# Autodesk Inventor assembly: 4_right_leg_true_final
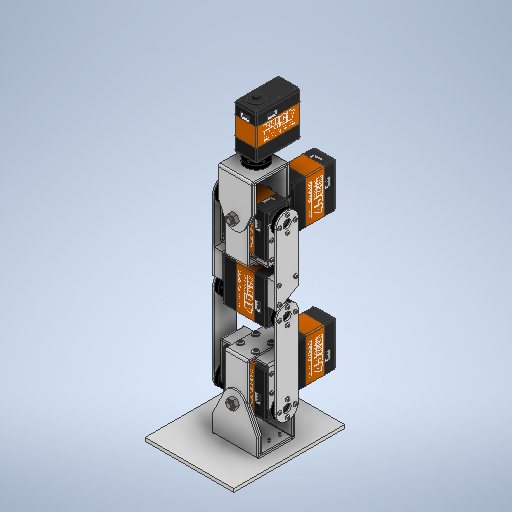
[picture p0: Inventor's stored thumbnail of the model, 512x512]
Saved by Autodesk Inventor 2026.1 (Build 301233000, 233)
## iProperties
Created: 2025-08-13
Part Number: 4_right_leg_true_final
Document SubType Name: Assembly
Designer: User
Author: User
## Documents named in this file (28)
- C:\Users\User\Documents\The Maverick's Files\College 3-3\로보인 프로젝트\RHp_Humanoid_ver1\Assembly\4_right_leg_true_final.iam
- C:\Users\User\Documents\The Maverick's Files\College 3-3\로보인 프로젝트\RHp_Humanoid_ver1\Part\HTD-45H, Horn\HTD-45H\HTD-45H.iam
- C:\Users\User\Documents\The Maverick's Files\College 3-3\로보인 프로젝트\RHp_Humanoid_ver1\Part\HTD-45H, Horn\Horn\Top Horn.ipt
- C:\Users\User\Documents\The Maverick's Files\College 3-3\로보인 프로젝트\RHp_Humanoid_ver1\Part\HTD-45H, Horn\Horn\Bottom Horn.ipt
- C:\Users\User\Documents\The Maverick's Files\College 3-3\로보인 프로젝트\RHp_Humanoid_ver1\Part\Frame\Leg\Right Leg\axis_7_supplement_frame.ipt
- C:\Users\User\Documents\The Maverick's Files\College 3-3\로보인 프로젝트\RHp_Humanoid_ver1\Part\Frame\Leg\Right Leg\axis_7_top_frame.ipt
- C:\Users\User\Documents\The Maverick's Files\College 3-3\로보인 프로젝트\RHp_Humanoid_ver1\Part\Frame\Leg\Right Leg\axis_8_bottom_frame.ipt
- C:\Users\User\Documents\The Maverick's Files\College 3-3\로보인 프로젝트\RHp_Humanoid_ver1\Part\Frame\Leg\Right Leg\axis_8_10_connector_frame_non_powered.ipt
- C:\Users\User\Documents\The Maverick's Files\College 3-3\로보인 프로젝트\RHp_Humanoid_ver1\Part\Frame\Leg\Right Leg\axis_8_10_connector_frame_powered.ipt
- C:\Users\User\Documents\The Maverick's Files\College 3-3\로보인 프로젝트\RHp_Humanoid_ver1\Part\Frame\Leg\Right Leg\axis_9_bottom_frame.ipt
- C:\Users\User\Documents\The Maverick's Files\College 3-3\로보인 프로젝트\RHp_Humanoid_ver1\Part\Frame\Leg\3D_printed_part_non_powered.ipt
- C:\Users\User\Documents\The Maverick's Files\College 3-3\로보인 프로젝트\RHp_Humanoid_ver1\Part\Frame\Leg\3D_printed_part_powered.ipt
- C:\Users\User\Documents\The Maverick's Files\College 3-3\로보인 프로젝트\RHp_Humanoid_ver1\Part\Frame\Leg\Right Leg\axis_10_11_connector_frame_non_powered.ipt
- C:\Users\User\Documents\The Maverick's Files\College 3-3\로보인 프로젝트\RHp_Humanoid_ver1\Part\Frame\Leg\Right Leg\axis_10_11_connector_frame_powered.ipt
- C:\Users\User\Documents\The Maverick's Files\College 3-3\로보인 프로젝트\RHp_Humanoid_ver1\Part\Frame\Leg\Right Leg\axis_11_top_frame.ipt
- C:\Users\User\Documents\The Maverick's Files\College 3-3\로보인 프로젝트\RHp_Humanoid_ver1\Part\Frame\Leg\Right Leg\axis_12_top_frame.ipt
- C:\Users\User\Documents\The Maverick's Files\College 3-3\로보인 프로젝트\RHp_Humanoid_ver1\Part\Frame\Leg\Right Leg\axis_12_bottom_frame(top).ipt
- C:\Users\User\Documents\The Maverick's Files\College 3-3\로보인 프로젝트\RHp_Humanoid_ver1\Part\Frame\Leg\Right Leg\axis_12_supplement_frame.ipt
- C:\Users\User\Documents\The Maverick's Files\College 3-3\로보인 프로젝트\RHp_Humanoid_ver1\Part\Frame\Leg\Right Leg\axis_12_bottom_frame(bottom).ipt
- C:\Users\User\Documents\The Maverick's Files\College 3-3\로보인 프로젝트\RHp_Humanoid_ver1\Part\Bolt, Bearing, Nut, Washer\볼트, 너트\볼트, 너트\M2x8접시.ipt
- C:\Users\User\Documents\The Maverick's Files\College 3-3\로보인 프로젝트\RHp_Humanoid_ver1\Part\Bolt, Bearing, Nut, Washer\볼트, 너트\볼트, 너트\M5x10 Bolt.ipt
- C:\Users\User\Documents\The Maverick's Files\College 3-3\로보인 프로젝트\RHp_Humanoid_ver1\Part\Bolt, Bearing, Nut, Washer\볼트, 너트\볼트, 너트\M5 Nylon Nut.ipt
- C:\Users\User\Documents\The Maverick's Files\College 3-3\로보인 프로젝트\RHp_Humanoid_ver1\Part\Bolt, Bearing, Nut, Washer\볼트, 너트\볼트, 너트\M3x6 Bolt.ipt
- C:\Users\User\Documents\The Maverick's Files\College 3-3\로보인 프로젝트\RHp_Humanoid_ver1\Part\Bolt, Bearing, Nut, Washer\볼트, 너트\볼트, 너트\M3 Nut.ipt
- C:\Users\User\Documents\The Maverick's Files\College 3-3\로보인 프로젝트\RHp_Humanoid_ver1\Part\Bolt, Bearing, Nut, Washer\볼트, 너트\볼트, 너트\M2x45 Bolt.ipt
- C:\Users\User\Documents\The Maverick's Files\College 3-3\로보인 프로젝트\RHp_Humanoid_ver1\Part\Bolt, Bearing, Nut, Washer\볼트, 너트\볼트, 너트\M2x12 Bolt.ipt
- C:\Users\User\Documents\The Maverick's Files\College 3-3\로보인 프로젝트\RHp_Humanoid_ver1\Part\Bolt, Bearing, Nut, Washer\볼트, 너트\볼트, 너트\M2x6 Bolt.ipt
- C:\Users\User\Documents\The Maverick's Files\College 3-3\로보인 프로젝트\RHp_Humanoid_ver1\Part\Bolt, Bearing, Nut, Washer\볼트, 너트\볼트, 너트\M2x4 Bolt.ipt
## Components (128 placed, 27 different names)
1. HTD-45H:1 [sub-assembly] — Rotational:1
2. Top Horn:1 — Rotational:1, Rigid:1
3. axis_7_top_frame:1 — Rigid:1, Rigid:2, Rigid:4, Rigid:31
4. axis_7_supplement_frame:1 — Rigid:2, Rigid:29, Rigid:89, Rigid:90, Rigid:91, Rigid:92, Rigid:93, Rigid:94, Rigid:95, Rigid:96
5. HTD-45H:2 [sub-assembly] — Rotational:2, Rigid:3
6. Top Horn:2 — Rigid:7
7. Bottom Horn:2 — Rotational:2, Rigid:8
8. axis_8_bottom_frame:1 — Rigid:3, Rigid:6, Rigid:37, Rigid:38, Rigid:39, Rigid:40, Rigid:71, Rigid:72, Rigid:73, Rigid:74, Rigid:75, Rigid:76, Rigid:77, Rigid:78, Rigid:79
9. axis_8_10_connector_frame_powered:1 — Rigid:7, Rigid:9, Rigid:49, Rigid:50, Rigid:51, Rigid:52, Rigid:53, Rigid:105, Rigid:106, Rigid:107, Rigid:108
10. axis_8_10_connector_frame_non_powered:1 — Rigid:8, Rigid:10, Rigid:54, Rigid:55, Rigid:56, Rigid:113, Rigid:114, Rigid:115, Rigid:116
11. HTD-45H:3 [sub-assembly] — Rotational:5, Rigid:5
12. Top Horn:3 — Rotational:5, Rigid:4
13. axis_9_bottom_frame:1 — Rigid:5, Rigid:6, Rigid:45, Rigid:46, Rigid:47, Rigid:48, Rigid:80, Rigid:81, Rigid:82, Rigid:83, Rigid:84
14. HTD-45H:4 [sub-assembly] — Rotational:6, Rotational:7, Rigid:11, Rigid:12
15. Top Horn:4 — Rotational:7, Rigid:13
16. Bottom Horn:4 — Rotational:6, Rigid:14
17. 3D_printed_part_powered:1 — Rigid:9, Rigid:11
18. 3D_printed_part_non_powered:1 — Rigid:10, Rigid:12
19. axis_10_11_connector_frame_powered:1 — Rigid:13, Rotational:10, Rigid:97, Rigid:98, Rigid:99, Rigid:100, Rigid:101, Rigid:102, Rigid:103, Rigid:104
20. axis_10_11_connector_frame_non_powered:1 — Rigid:14, Rigid:17, Rigid:109, Rigid:110, Rigid:111, Rigid:112, Rigid:117, Rigid:118, Rigid:119, Rigid:120
21. HTD-45H:5 [sub-assembly] — Rotational:8, Rigid:16, Rigid:15
22. Top Horn:5 — Rigid:16, Rotational:10
23. Bottom Horn:5 — Rotational:8, Rigid:17
24. axis_11_top_frame:1 — Rigid:15, Rigid:19, Rigid:41, Rigid:42, Rigid:43, Rigid:44, Rigid:57, Rigid:58, Rigid:59, Rigid:60, Rigid:61, Rigid:62, Rigid:63, Rigid:64, Rigid:65
25. HTD-45H:6 [sub-assembly] — Rotational:11, Rigid:18
26. Top Horn:6 — Rotational:11, Rigid:20
27. axis_12_top_frame:1 — Rigid:18, Rigid:19, Rigid:33, Rigid:34, Rigid:35, Rigid:36, Rigid:66, Rigid:67, Rigid:68, Rigid:69, Rigid:70
28. axis_12_supplement_frame:1 — Rigid:21, Rigid:30, Rigid:85, Rigid:86, Rigid:87, Rigid:88
29. axis_12_bottom_frame(top):1 — Rigid:20, Rigid:21, Rigid:22, Rigid:32
30. axis_12_bottom_frame(bottom):1 — Rigid:22, Rigid:23, Rigid:24, Rigid:25, Rigid:26, Rigid:27, Rigid:28
31. M2x4 Bolt:1 — Rigid:97
32. M2x4 Bolt:2 — Rigid:98
33. M2x4 Bolt:3 — Rigid:99
34. M2x4 Bolt:4 — Rigid:100
35. M2x4 Bolt:5 — Rigid:101
36. M2x4 Bolt:6 — Rigid:102
37. M2x4 Bolt:7 — Rigid:103
38. M2x4 Bolt:8 — Rigid:104
39. M2x4 Bolt:9 — Rigid:105
40. M2x4 Bolt:10 — Rigid:106
41. M2x4 Bolt:11 — Rigid:107
42. M2x4 Bolt:12 — Rigid:108
43. M2x4 Bolt:13 — Rigid:113
44. M2x4 Bolt:14 — Rigid:114
45. M2x4 Bolt:15 — Rigid:115
46. M2x4 Bolt:16 — Rigid:116
47. M2x4 Bolt:17 — Rigid:117
48. M2x4 Bolt:18 — Rigid:118
49. M2x4 Bolt:19 — Rigid:119
50. M2x4 Bolt:20 — Rigid:120
51. M2x4 Bolt:21 — Rigid:109
52. M2x4 Bolt:22 — Rigid:110
53. M2x4 Bolt:23 — Rigid:111
54. M2x4 Bolt:24 — Rigid:112
55. M2x6 Bolt:1 — Rigid:57
56. M2x6 Bolt:2 — Rigid:58
57. M2x6 Bolt:3 — Rigid:59
58. M2x6 Bolt:4 — Rigid:60
59. M2x6 Bolt:5 — Rigid:61
60. M2x6 Bolt:6 — Rigid:62
61. M2x6 Bolt:7 — Rigid:63
62. M2x6 Bolt:8 — Rigid:64
63. M2x6 Bolt:9 — Rigid:65
64. M2x6 Bolt:10 — Rigid:66
65. M2x6 Bolt:11 — Rigid:67
66. M2x6 Bolt:12 — Rigid:68
67. M2x6 Bolt:13 — Rigid:69
68. M2x6 Bolt:14 — Rigid:70
69. M2x6 Bolt:15 — Rigid:71
70. M2x6 Bolt:16 — Rigid:72
71. M2x6 Bolt:17 — Rigid:73
72. M2x6 Bolt:18 — Rigid:74
73. M2x6 Bolt:19 — Rigid:75
74. M2x6 Bolt:20 — Rigid:76
75. M2x6 Bolt:21 — Rigid:77
76. M2x6 Bolt:22 — Rigid:78
77. M2x6 Bolt:23 — Rigid:79
78. M2x6 Bolt:24 — Rigid:80
79. M2x6 Bolt:25 — Rigid:81
80. M2x6 Bolt:26 — Rigid:82
81. M2x6 Bolt:27 — Rigid:83
82. M2x6 Bolt:28 — Rigid:84
83. M2x6 Bolt:29 — Rigid:85
84. M2x6 Bolt:30 — Rigid:86
85. M2x6 Bolt:31 — Rigid:87
86. M2x6 Bolt:32 — Rigid:88
87. M2x6 Bolt:33 — Rigid:89
88. M2x6 Bolt:34 — Rigid:90
89. M2x6 Bolt:35 — Rigid:91
90. M2x6 Bolt:36 — Rigid:92
91. M2x6 Bolt:37 — Rigid:93
92. M2x6 Bolt:38 — Rigid:94
93. M2x6 Bolt:39 — Rigid:95
94. M2x6 Bolt:40 — Rigid:96
95. M2x8접시:1 — Rigid:23
96. M2x8접시:2 — Rigid:24
97. M2x8접시:3 — Rigid:25
98. M2x8접시:4 — Rigid:26
99. M2x8접시:5 — Rigid:27
100. M2x8접시:6 — Rigid:28
101. M2x12 Bolt:1 — Rigid:51
102. M2x12 Bolt:2 — Rigid:52
103. M2x12 Bolt:3 — Rigid:53
104. M2x12 Bolt:4 — Rigid:54
105. M2x12 Bolt:5 — Rigid:55
106. M2x12 Bolt:6 — Rigid:56
107. M2x45 Bolt:1 — Rigid:49
108. M2x45 Bolt:2 — Rigid:50
109. M3x6 Bolt:1 — Rigid:33
110. M3x6 Bolt:2 — Rigid:34
111. M3x6 Bolt:3 — Rigid:35
112. M3x6 Bolt:4 — Rigid:36
113. M3x6 Bolt:5 — Rigid:37
114. M3x6 Bolt:6 — Rigid:38
115. M3x6 Bolt:7 — Rigid:39
116. M3x6 Bolt:8 — Rigid:40
117. M3 Nut:1 — Rigid:41
118. M3 Nut:2 — Rigid:42
119. M3 Nut:3 — Rigid:43
120. M3 Nut:4 — Rigid:44
121. M3 Nut:5 — Rigid:45
122. M3 Nut:6 — Rigid:46
123. M3 Nut:7 — Rigid:47
124. M3 Nut:8 — Rigid:48
125. M5x10 Bolt:1 — Rigid:29
126. M5x10 Bolt:2 — Rigid:30
127. M5 Nylon Nut:1 — Rigid:32
128. M5 Nylon Nut:2 — Rigid:31
## Relationships (128: WeldJoint 120, RevoluteJoint 8)
- Rotational:1 [RevoluteJoint]: HTD-45H:1 ↔ Top Horn:1
- Rigid:1 [WeldJoint]: Top Horn:1 ↔ axis_7_top_frame:1
- Rigid:2 [WeldJoint]: axis_7_top_frame:1 ↔ axis_7_supplement_frame:1
- Rotational:2 [RevoluteJoint]: HTD-45H:2 ↔ Bottom Horn:2
- Rigid:3 [WeldJoint]: HTD-45H:2 ↔ axis_8_bottom_frame:1
- Rotational:5 [RevoluteJoint]: HTD-45H:3 ↔ Top Horn:3
- Rigid:4 [WeldJoint]: axis_7_top_frame:1 ↔ Top Horn:3
- Rigid:5 [WeldJoint]: HTD-45H:3 ↔ axis_9_bottom_frame:1
- Rigid:6 [WeldJoint]: axis_8_bottom_frame:1 ↔ axis_9_bottom_frame:1
- Rigid:7 [WeldJoint]: Top Horn:2 ↔ axis_8_10_connector_frame_powered:1
- Rigid:8 [WeldJoint]: Bottom Horn:2 ↔ axis_8_10_connector_frame_non_powered:1
- Rigid:9 [WeldJoint]: axis_8_10_connector_frame_powered:1 ↔ 3D_printed_part_powered:1
- Rigid:10 [WeldJoint]: axis_8_10_connector_frame_non_powered:1 ↔ 3D_printed_part_non_powered:1
- Rotational:6 [RevoluteJoint]: HTD-45H:4 ↔ Bottom Horn:4
- Rotational:7 [RevoluteJoint]: HTD-45H:4 ↔ Top Horn:4
- Rigid:11 [WeldJoint]: HTD-45H:4 ↔ 3D_printed_part_powered:1
- Rigid:12 [WeldJoint]: HTD-45H:4 ↔ 3D_printed_part_non_powered:1
- Rigid:13 [WeldJoint]: Top Horn:4 ↔ axis_10_11_connector_frame_powered:1
- Rigid:14 [WeldJoint]: Bottom Horn:4 ↔ axis_10_11_connector_frame_non_powered:1
- Rotational:8 [RevoluteJoint]: HTD-45H:5 ↔ Bottom Horn:5
- Rigid:16 [WeldJoint]: HTD-45H:5 ↔ Top Horn:5
- Rigid:15 [WeldJoint]: HTD-45H:5 ↔ axis_11_top_frame:1
- Rotational:10 [RevoluteJoint]: axis_10_11_connector_frame_powered:1 ↔ Top Horn:5
- Rigid:17 [WeldJoint]: axis_10_11_connector_frame_non_powered:1 ↔ Bottom Horn:5
- Rotational:11 [RevoluteJoint]: HTD-45H:6 ↔ Top Horn:6
- Rigid:18 [WeldJoint]: HTD-45H:6 ↔ axis_12_top_frame:1
- Rigid:19 [WeldJoint]: axis_11_top_frame:1 ↔ axis_12_top_frame:1
- Rigid:20 [WeldJoint]: Top Horn:6 ↔ axis_12_bottom_frame(top):1
- Rigid:21 [WeldJoint]: axis_12_supplement_frame:1 ↔ axis_12_bottom_frame(top):1
- Rigid:22 [WeldJoint]: axis_12_bottom_frame(top):1 ↔ axis_12_bottom_frame(bottom):1
- Rigid:23 [WeldJoint]: axis_12_bottom_frame(bottom):1 ↔ M2x8접시:1
- Rigid:24 [WeldJoint]: axis_12_bottom_frame(bottom):1 ↔ M2x8접시:2
- Rigid:25 [WeldJoint]: axis_12_bottom_frame(bottom):1 ↔ M2x8접시:3
- Rigid:26 [WeldJoint]: axis_12_bottom_frame(bottom):1 ↔ M2x8접시:4
- Rigid:27 [WeldJoint]: axis_12_bottom_frame(bottom):1 ↔ M2x8접시:5
- Rigid:28 [WeldJoint]: axis_12_bottom_frame(bottom):1 ↔ M2x8접시:6
- Rigid:29 [WeldJoint]: axis_7_supplement_frame:1 ↔ M5x10 Bolt:1
- Rigid:30 [WeldJoint]: axis_12_supplement_frame:1 ↔ M5x10 Bolt:2
- Rigid:31 [WeldJoint]: axis_7_top_frame:1 ↔ M5 Nylon Nut:2
- Rigid:32 [WeldJoint]: axis_12_bottom_frame(top):1 ↔ M5 Nylon Nut:1
- Rigid:33 [WeldJoint]: axis_12_top_frame:1 ↔ M3x6 Bolt:1
- Rigid:34 [WeldJoint]: axis_12_top_frame:1 ↔ M3x6 Bolt:2
- Rigid:35 [WeldJoint]: axis_12_top_frame:1 ↔ M3x6 Bolt:3
- Rigid:36 [WeldJoint]: axis_12_top_frame:1 ↔ M3x6 Bolt:4
- Rigid:37 [WeldJoint]: axis_8_bottom_frame:1 ↔ M3x6 Bolt:5
- Rigid:38 [WeldJoint]: axis_8_bottom_frame:1 ↔ M3x6 Bolt:6
- Rigid:39 [WeldJoint]: axis_8_bottom_frame:1 ↔ M3x6 Bolt:7
- Rigid:40 [WeldJoint]: axis_8_bottom_frame:1 ↔ M3x6 Bolt:8
- Rigid:41 [WeldJoint]: axis_11_top_frame:1 ↔ M3 Nut:1
- Rigid:42 [WeldJoint]: axis_11_top_frame:1 ↔ M3 Nut:2
- Rigid:43 [WeldJoint]: axis_11_top_frame:1 ↔ M3 Nut:3
- Rigid:44 [WeldJoint]: axis_11_top_frame:1 ↔ M3 Nut:4
- Rigid:45 [WeldJoint]: axis_9_bottom_frame:1 ↔ M3 Nut:5
- Rigid:46 [WeldJoint]: axis_9_bottom_frame:1 ↔ M3 Nut:6
- Rigid:47 [WeldJoint]: axis_9_bottom_frame:1 ↔ M3 Nut:7
- Rigid:48 [WeldJoint]: axis_9_bottom_frame:1 ↔ M3 Nut:8
- Rigid:49 [WeldJoint]: axis_8_10_connector_frame_powered:1 ↔ M2x45 Bolt:1
- Rigid:50 [WeldJoint]: axis_8_10_connector_frame_powered:1 ↔ M2x45 Bolt:2
- Rigid:51 [WeldJoint]: axis_8_10_connector_frame_powered:1 ↔ M2x12 Bolt:1
- Rigid:52 [WeldJoint]: axis_8_10_connector_frame_powered:1 ↔ M2x12 Bolt:2
- Rigid:53 [WeldJoint]: axis_8_10_connector_frame_powered:1 ↔ M2x12 Bolt:3
- Rigid:54 [WeldJoint]: axis_8_10_connector_frame_non_powered:1 ↔ M2x12 Bolt:4
- Rigid:55 [WeldJoint]: axis_8_10_connector_frame_non_powered:1 ↔ M2x12 Bolt:5
- Rigid:56 [WeldJoint]: axis_8_10_connector_frame_non_powered:1 ↔ M2x12 Bolt:6
- Rigid:57 [WeldJoint]: axis_11_top_frame:1 ↔ M2x6 Bolt:1
- Rigid:58 [WeldJoint]: axis_11_top_frame:1 ↔ M2x6 Bolt:2
- Rigid:59 [WeldJoint]: axis_11_top_frame:1 ↔ M2x6 Bolt:3
- Rigid:60 [WeldJoint]: axis_11_top_frame:1 ↔ M2x6 Bolt:4
- Rigid:61 [WeldJoint]: axis_11_top_frame:1 ↔ M2x6 Bolt:5
- Rigid:62 [WeldJoint]: axis_11_top_frame:1 ↔ M2x6 Bolt:6
- Rigid:63 [WeldJoint]: axis_11_top_frame:1 ↔ M2x6 Bolt:7
- Rigid:64 [WeldJoint]: axis_11_top_frame:1 ↔ M2x6 Bolt:8
- Rigid:65 [WeldJoint]: axis_11_top_frame:1 ↔ M2x6 Bolt:9
- Rigid:66 [WeldJoint]: axis_12_top_frame:1 ↔ M2x6 Bolt:10
- Rigid:67 [WeldJoint]: axis_12_top_frame:1 ↔ M2x6 Bolt:11
- Rigid:68 [WeldJoint]: axis_12_top_frame:1 ↔ M2x6 Bolt:12
- Rigid:69 [WeldJoint]: axis_12_top_frame:1 ↔ M2x6 Bolt:13
- Rigid:70 [WeldJoint]: axis_12_top_frame:1 ↔ M2x6 Bolt:14
- Rigid:71 [WeldJoint]: axis_8_bottom_frame:1 ↔ M2x6 Bolt:15
- Rigid:72 [WeldJoint]: axis_8_bottom_frame:1 ↔ M2x6 Bolt:16
- Rigid:73 [WeldJoint]: axis_8_bottom_frame:1 ↔ M2x6 Bolt:17
- Rigid:74 [WeldJoint]: axis_8_bottom_frame:1 ↔ M2x6 Bolt:18
- Rigid:75 [WeldJoint]: axis_8_bottom_frame:1 ↔ M2x6 Bolt:19
- Rigid:76 [WeldJoint]: axis_8_bottom_frame:1 ↔ M2x6 Bolt:20
- Rigid:77 [WeldJoint]: axis_8_bottom_frame:1 ↔ M2x6 Bolt:21
- Rigid:78 [WeldJoint]: axis_8_bottom_frame:1 ↔ M2x6 Bolt:22
- Rigid:79 [WeldJoint]: axis_8_bottom_frame:1 ↔ M2x6 Bolt:23
- Rigid:80 [WeldJoint]: axis_9_bottom_frame:1 ↔ M2x6 Bolt:24
- Rigid:81 [WeldJoint]: axis_9_bottom_frame:1 ↔ M2x6 Bolt:25
- Rigid:82 [WeldJoint]: axis_9_bottom_frame:1 ↔ M2x6 Bolt:26
- Rigid:83 [WeldJoint]: axis_9_bottom_frame:1 ↔ M2x6 Bolt:27
- Rigid:84 [WeldJoint]: axis_9_bottom_frame:1 ↔ M2x6 Bolt:28
- Rigid:85 [WeldJoint]: axis_12_supplement_frame:1 ↔ M2x6 Bolt:29
- Rigid:86 [WeldJoint]: axis_12_supplement_frame:1 ↔ M2x6 Bolt:30
- Rigid:87 [WeldJoint]: axis_12_supplement_frame:1 ↔ M2x6 Bolt:31
- Rigid:88 [WeldJoint]: axis_12_supplement_frame:1 ↔ M2x6 Bolt:32
- Rigid:89 [WeldJoint]: axis_7_supplement_frame:1 ↔ M2x6 Bolt:33
- Rigid:90 [WeldJoint]: axis_7_supplement_frame:1 ↔ M2x6 Bolt:34
- Rigid:91 [WeldJoint]: axis_7_supplement_frame:1 ↔ M2x6 Bolt:35
- Rigid:92 [WeldJoint]: axis_7_supplement_frame:1 ↔ M2x6 Bolt:36
- Rigid:93 [WeldJoint]: axis_7_supplement_frame:1 ↔ M2x6 Bolt:37
- Rigid:94 [WeldJoint]: axis_7_supplement_frame:1 ↔ M2x6 Bolt:38
- Rigid:95 [WeldJoint]: axis_7_supplement_frame:1 ↔ M2x6 Bolt:39
- Rigid:96 [WeldJoint]: axis_7_supplement_frame:1 ↔ M2x6 Bolt:40
- Rigid:97 [WeldJoint]: axis_10_11_connector_frame_powered:1 ↔ M2x4 Bolt:1
- Rigid:98 [WeldJoint]: axis_10_11_connector_frame_powered:1 ↔ M2x4 Bolt:2
- Rigid:99 [WeldJoint]: axis_10_11_connector_frame_powered:1 ↔ M2x4 Bolt:3
- Rigid:100 [WeldJoint]: axis_10_11_connector_frame_powered:1 ↔ M2x4 Bolt:4
- Rigid:101 [WeldJoint]: axis_10_11_connector_frame_powered:1 ↔ M2x4 Bolt:5
- Rigid:102 [WeldJoint]: axis_10_11_connector_frame_powered:1 ↔ M2x4 Bolt:6
- Rigid:103 [WeldJoint]: axis_10_11_connector_frame_powered:1 ↔ M2x4 Bolt:7
- Rigid:104 [WeldJoint]: axis_10_11_connector_frame_powered:1 ↔ M2x4 Bolt:8
- Rigid:105 [WeldJoint]: axis_8_10_connector_frame_powered:1 ↔ M2x4 Bolt:9
- Rigid:106 [WeldJoint]: axis_8_10_connector_frame_powered:1 ↔ M2x4 Bolt:10
- Rigid:107 [WeldJoint]: axis_8_10_connector_frame_powered:1 ↔ M2x4 Bolt:11
- Rigid:108 [WeldJoint]: axis_8_10_connector_frame_powered:1 ↔ M2x4 Bolt:12
- Rigid:109 [WeldJoint]: axis_10_11_connector_frame_non_powered:1 ↔ M2x4 Bolt:21
- Rigid:110 [WeldJoint]: axis_10_11_connector_frame_non_powered:1 ↔ M2x4 Bolt:22
- Rigid:111 [WeldJoint]: axis_10_11_connector_frame_non_powered:1 ↔ M2x4 Bolt:23
- Rigid:112 [WeldJoint]: axis_10_11_connector_frame_non_powered:1 ↔ M2x4 Bolt:24
- Rigid:113 [WeldJoint]: axis_8_10_connector_frame_non_powered:1 ↔ M2x4 Bolt:13
- Rigid:114 [WeldJoint]: axis_8_10_connector_frame_non_powered:1 ↔ M2x4 Bolt:14
- Rigid:115 [WeldJoint]: axis_8_10_connector_frame_non_powered:1 ↔ M2x4 Bolt:15
- Rigid:116 [WeldJoint]: axis_8_10_connector_frame_non_powered:1 ↔ M2x4 Bolt:16
- Rigid:117 [WeldJoint]: axis_10_11_connector_frame_non_powered:1 ↔ M2x4 Bolt:17
- Rigid:118 [WeldJoint]: axis_10_11_connector_frame_non_powered:1 ↔ M2x4 Bolt:18
- Rigid:119 [WeldJoint]: axis_10_11_connector_frame_non_powered:1 ↔ M2x4 Bolt:19
- Rigid:120 [WeldJoint]: axis_10_11_connector_frame_non_powered:1 ↔ M2x4 Bolt:20
